# Autodesk Inventor assembly: ShoulderConnectorSplit
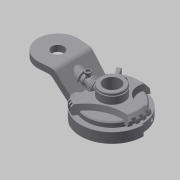
[picture p0: Inventor's stored thumbnail of the model, 180x180]
Saved by Autodesk Inventor 2015 SP1 (Build 190203100, 203)
## iProperties
Created: 2015-12-02
Part Number: ShoulderConnectorSplit
Document SubType Name: Assembly
Designer: Val
Author: Val
## Documents named in this file (3)
- C:\Users\Val\Desktop\ExoGit\elysium-max-exoskeleton\src\Assemblies\ShoulderConnector.iam
- C:\Users\Val\Desktop\ExoGit\elysium-max-exoskeleton\src\ShoulderConnectorSplitBody.ipt
- C:\Users\Val\Desktop\ExoGit\elysium-max-exoskeleton\src\ShoulderConnectorSplitHead.ipt
## Components (2 placed, 2 different names)
1. ShoulderConnectorSplitBody:1 — Mate:1, Mate:2
2. ShoulderConnectorSplitHead:1 — Mate:1, Mate:2
## Relationships (2: Mate 2)
- Mate:1: ShoulderConnectorSplitBody:1 ↔ ShoulderConnectorSplitHead:1
- Mate:2: ShoulderConnectorSplitBody:1 ↔ ShoulderConnectorSplitHead:1
